# Autodesk Inventor assembly: Button Box Assembly
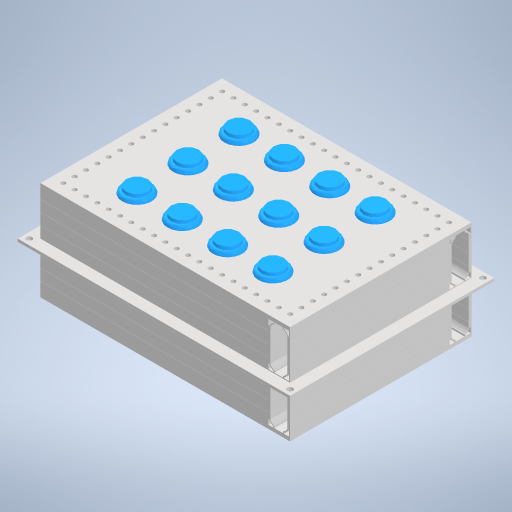
[picture p0: Inventor's stored thumbnail of the model, 512x512]
Saved by Autodesk Inventor 2023.4 (Build 274418000, 418)
## iProperties
Created: 2023-12-24
Part Number: Button Box Assembly
Document SubType Name: Assembly
Designer: amrom
Author: amrom
## Documents named in this file (7)
- C:\Users\amrom\OneDrive\Desktop\Driver's station\Button Box\Button Box Assembly.iam
- C:\Users\amrom\OneDrive\Desktop\Driver's station\Button Box\7in side.ipt
- C:\Users\amrom\OneDrive\Desktop\Driver's station\Button Box\8in top.ipt
- C:\Users\amrom\OneDrive\Desktop\Driver's station\Button Box\Middle plate.ipt
- C:\Users\amrom\OneDrive\Desktop\Driver's station\Button Box\Bottom Plate.ipt
- C:\Users\amrom\OneDrive\Desktop\Driver's station\Button Box\Top Plate.ipt
- C:\Users\amrom\OneDrive\Desktop\Driver's station\Arcade Button30mm.ipt
## Components (23 placed, 6 different names)
1. 7in side:1 — Flush:3, Flush:4, Flush:5, Mate:2, Flush:6, Flush:7, Mate:3, Mate:5, Flush:10, Flush:18, Mate:12
2. 7in side:2 — Mate:4, Flush:8, Flush:9, Flush:13, Mate:11
3. 8in top:1 — Flush:6, Flush:7, Mate:3, Mate:4, Flush:8, Flush:12
4. 8in top:2 — Flush:3, Flush:4, Flush:5, Mate:2, Flush:9, Mate:6, Flush:15, Flush:19
5. Middle plate:1 — Mate:5, Flush:10, Mate:6, Flush:11, Mate:7, Flush:14, Mate:8, Mate:9, Flush:16, Flush:17, Mate:10
6. 8in top:3 — Flush:11, Mate:7, Flush:12
7. 8in top:4 — Mate:9, Flush:15, Flush:16, Mate:14
8. 7in side:3 — Flush:13, Flush:14, Mate:8, Mate:13, Flush:20
9. 7in side:4 — Flush:17, Mate:10, Flush:18
10. Bottom Plate:1 — Mate:11, Mate:12, Flush:19
11. Top Plate:1 — Mate:13, Flush:20, Mate:14, Mate:15, Mate:16, Mate:17, Mate:18, Mate:19, Mate:20, Mate:21, Mate:22, Mate:23, Mate:24, Mate:25, Mate:26, Mate:27, Mate:28, Mate:29, Mate:30, Mate:31, Mate:32, Mate:33, Mate:34, Mate:35, Mate:36, Mate:37, Mate:38
12. Arcade Button30mm:2 — Mate:15, Mate:16
13. Arcade Button30mm:3 — Mate:17, Mate:18
14. Arcade Button30mm:4 — Mate:19, Mate:20
15. Arcade Button30mm:5 — Mate:21, Mate:22
16. Arcade Button30mm:6 — Mate:25, Mate:26
17. Arcade Button30mm:7 — Mate:35, Mate:36
18. Arcade Button30mm:8 — Mate:33, Mate:34
19. Arcade Button30mm:9 — Mate:23, Mate:24
20. Arcade Button30mm:10 — Mate:31, Mate:32
21. Arcade Button30mm:11 — Mate:28, Mate:29
22. Arcade Button30mm:12 — Mate:27, Mate:30
23. Arcade Button30mm:13 — Mate:37, Mate:38
## Relationships (55: Mate 37, Flush 18)
- Flush:3: 7in side:1 ↔ 8in top:2
- Flush:4: 7in side:1 ↔ 8in top:2
- Flush:5: 7in side:1 ↔ 8in top:2
- Mate:2: 7in side:1 ↔ 8in top:2
- Flush:6: 7in side:1 ↔ 8in top:1
- Flush:7: 7in side:1 ↔ 8in top:1
- Mate:3: 7in side:1 ↔ 8in top:1
- Mate:4: 7in side:2 ↔ 8in top:1
- Flush:8: 7in side:2 ↔ 8in top:1
- Flush:9: 7in side:2 ↔ 8in top:2
- Mate:5: 7in side:1 ↔ Middle plate:1
- Flush:10: 7in side:1 ↔ Middle plate:1
- Mate:6: 8in top:2 ↔ Middle plate:1
- Flush:11: Middle plate:1 ↔ 8in top:3
- Mate:7: Middle plate:1 ↔ 8in top:3
- Flush:12: 8in top:1 ↔ 8in top:3
- Flush:13: 7in side:2 ↔ 7in side:3
- Flush:14: Middle plate:1 ↔ 7in side:3
- Mate:8: Middle plate:1 ↔ 7in side:3
- Mate:9: Middle plate:1 ↔ 8in top:4
- Flush:15: 8in top:2 ↔ 8in top:4
- Flush:16: Middle plate:1 ↔ 8in top:4
- Flush:17: Middle plate:1 ↔ 7in side:4
- Mate:10: Middle plate:1 ↔ 7in side:4
- Flush:18: 7in side:1 ↔ 7in side:4
- Mate:11: 7in side:2 ↔ Bottom Plate:1
- Mate:12: 7in side:1 ↔ Bottom Plate:1
- Flush:19: 8in top:2 ↔ Bottom Plate:1
- Mate:13: 7in side:3 ↔ Top Plate:1
- Flush:20: 7in side:3 ↔ Top Plate:1
- Mate:14: 8in top:4 ↔ Top Plate:1
- Mate:15: Top Plate:1 ↔ Arcade Button30mm:2
- Mate:16: Top Plate:1 ↔ Arcade Button30mm:2
- Mate:17: Top Plate:1 ↔ Arcade Button30mm:3
- Mate:18: Top Plate:1 ↔ Arcade Button30mm:3
- Mate:19: Top Plate:1 ↔ Arcade Button30mm:4
- Mate:20: Top Plate:1 ↔ Arcade Button30mm:4
- Mate:21: Top Plate:1 ↔ Arcade Button30mm:5
- Mate:22: Top Plate:1 ↔ Arcade Button30mm:5
- Mate:23: Top Plate:1 ↔ Arcade Button30mm:9
- Mate:24: Top Plate:1 ↔ Arcade Button30mm:9
- Mate:25: Top Plate:1 ↔ Arcade Button30mm:6
- Mate:26: Top Plate:1 ↔ Arcade Button30mm:6
- Mate:27: Top Plate:1 ↔ Arcade Button30mm:12
- Mate:28: Top Plate:1 ↔ Arcade Button30mm:11
- Mate:29: Top Plate:1 ↔ Arcade Button30mm:11
- Mate:30: Top Plate:1 ↔ Arcade Button30mm:12
- Mate:31: Top Plate:1 ↔ Arcade Button30mm:10
- Mate:32: Top Plate:1 ↔ Arcade Button30mm:10
- Mate:33: Top Plate:1 ↔ Arcade Button30mm:8
- Mate:34: Top Plate:1 ↔ Arcade Button30mm:8
- Mate:35: Top Plate:1 ↔ Arcade Button30mm:7
- Mate:36: Top Plate:1 ↔ Arcade Button30mm:7
- Mate:37: Top Plate:1 ↔ Arcade Button30mm:13
- Mate:38: Top Plate:1 ↔ Arcade Button30mm:13
